# Autodesk Inventor assembly: Mount_LCD
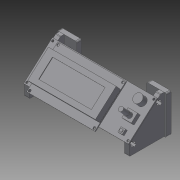
[picture p0: Inventor's stored thumbnail of the model, 180x180]
Saved by Autodesk Inventor 2014 (Build 180170000, 170)
## iProperties
Created: 2014-10-27
Part Number: Mount_LCD
Document SubType Name: Assembly
Designer: ThatOtherGuy
Author: ThatOtherGuy
## Documents named in this file (7)
- C:\Users\ThatOtherGuy\Documents\Inventor\KosselCNC1515\Mounts\Mount_LCD.iam
- C:\Users\ThatOtherGuy\Documents\Inventor\KosselCNC1515\Mounts\Mount_LCD_Back.ipt
- C:\Users\ThatOtherGuy\Documents\Inventor\KosselCNC1515\Mounts\Mount_LCD_End.ipt
- C:\Users\ThatOtherGuy\Documents\Inventor\KosselCNC1515\Mounts\RepRapDiscount-SmartController\RepRapDiscount_SmartController.ipt
- C:\Users\ThatOtherGuy\Documents\Inventor\KosselCNC1515\Mounts\Mount_LCD_End_SD.ipt
- C:\Users\ThatOtherGuy\Documents\Inventor\Content Center Files\R2014\en-US\ANSI B18.3.1M(1)\ANSI B18.3.1M - M3x0.5 x 10(2).ipt
- C:\Users\ThatOtherGuy\Documents\Inventor\Content Center Files\R2014\en-US\DIN 562\DIN 562 - M3 x 5.5.ipt
## Components (8 placed, 6 different names)
1. Mount_LCD_Back:1 — Mate:1, Mate:2, Mate:3, Mate:4, Mate:5, Mate:6, Insert:1, Insert:2, Insert:3, Insert:4
2. Mount_LCD_End:1 — Mate:1, Mate:2, Mate:3, Mate:7, Flush:1
3. Mount_LCD_End_SD:1 — Mate:4, Mate:5, Mate:6, Mate:8
4. RepRapDiscount_SmartController:1 — Mate:7, Flush:1, Mate:8
5. Broached Socket Head Cap Screw - Metric M3x0.5 x 10:1 — Insert:1
6. Broached Socket Head Cap Screw - Metric M3x0.5 x 10:2 — Insert:2
7. DIN 562 M3:1 — Insert:3
8. DIN 562 M3:2 — Insert:4
## Relationships (13: Mate 8, Insert 4, Flush 1)
- Mate:1: Mount_LCD_Back:1 ↔ Mount_LCD_End:1
- Mate:2: Mount_LCD_Back:1 ↔ Mount_LCD_End:1
- Mate:3: Mount_LCD_Back:1 ↔ Mount_LCD_End:1
- Mate:4: Mount_LCD_Back:1 ↔ Mount_LCD_End_SD:1
- Mate:5: Mount_LCD_Back:1 ↔ Mount_LCD_End_SD:1
- Mate:6: Mount_LCD_Back:1 ↔ Mount_LCD_End_SD:1
- Mate:7: Mount_LCD_End:1 ↔ RepRapDiscount_SmartController:1
- Flush:1: Mount_LCD_End:1 ↔ RepRapDiscount_SmartController:1
- Mate:8: Mount_LCD_End_SD:1 ↔ RepRapDiscount_SmartController:1
- Insert:1: Mount_LCD_Back:1 ↔ Broached Socket Head Cap Screw - Metric M3x0.5 x 10:1
- Insert:2: Mount_LCD_Back:1 ↔ Broached Socket Head Cap Screw - Metric M3x0.5 x 10:2
- Insert:3: Mount_LCD_Back:1 ↔ DIN 562 M3:1
- Insert:4: Mount_LCD_Back:1 ↔ DIN 562 M3:2
